# Autodesk Inventor assembly: centre wing
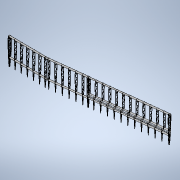
[picture p0: Inventor's stored thumbnail of the model, 180x180]
Saved by Autodesk Inventor 2022 (Build 260153000, 153)
## iProperties
Created: 2021-03-09
Part Number: centre wing
Document SubType Name: Assembly
Designer: Ferdinand Hubbard
Author: Ferdinand Hubbard
## Documents named in this file (15)
- C:\Users\Ferdinand Hubbard\Desktop\solarplane\cad\left wing section.iam
- C:\Users\Ferdinand Hubbard\Desktop\solarplane\cad\tubes\normal tubes\18mm tube.ipt
- C:\Users\Ferdinand Hubbard\Desktop\solarplane\cad\airfoils\full airfoil\full airfoil blueprint 19 mm.ipt
- C:\Users\Ferdinand Hubbard\Desktop\solarplane\cad\tubes\normal tubes\angle connector 19 mm.ipt
- C:\Users\Ferdinand Hubbard\Desktop\solarplane\cad\tubes\pre-aileron tubes\angle connector 19 mm.ipt
- C:\Users\Ferdinand Hubbard\Desktop\solarplane\cad\airfoils\full airfoil adjacent to aileron\full adjacent to aileron airfoil 19 mm big hole.ipt
- C:\Users\Ferdinand Hubbard\Desktop\solarplane\cad\tubes\normal tubes\15mm tube.ipt
- C:\Users\Ferdinand Hubbard\Desktop\solarplane\cad\tubes\normal tubes\7mm tube.ipt
- C:\Users\Ferdinand Hubbard\Desktop\solarplane\cad\tubes\normal tubes\straight connector aileron spar.ipt
- C:\Users\Ferdinand Hubbard\Desktop\solarplane\cad\airfoils\front half aileron\front half airfoil 16 mm.ipt
- C:\Users\Ferdinand Hubbard\Desktop\solarplane\cad\airfoils\full airfoil adjacent to aileron\full adjacent to aileron airfoil 19 mm small hole.ipt
- C:\Users\Ferdinand Hubbard\Desktop\solarplane\cad\airfoils\front half aileron\front half airfoil 19 mm.ipt
- C:\Users\Ferdinand Hubbard\Desktop\solarplane\cad\airfoils\back half aileron\back half aileron airfoil 19mm.ipt
- C:\Users\Ferdinand Hubbard\Desktop\solarplane\cad\tubes\back aileron tubes\18mm tube.ipt
- C:\Users\Ferdinand Hubbard\Desktop\solarplane\cad\tubes\back aileron tubes\15mm tube.ipt
## Components (57 placed, 11 different names)
1. 18mm tube:1 — Angle:2, Mate:10, Flush:2, Mate:25, Mate:26
2. 18mm tube:2 — Angle:1, Mate:11, Flush:1, Flush:3, Mate:27, Mate:28
3. full airfoil blueprint 19 mm:2 — Mate:1, Mate:2, Mate:3, Angle:1, Angle:2, Mate:10, Mate:11, Flush:1, Flush:2, Mate:21, Mate:22
4. full airfoil blueprint 19 mm:3 — Mate:1, Mate:2, Mate:3, Mate:7, Mate:8, Mate:9
5. full airfoil blueprint 19 mm:4 — Mate:7, Mate:8, Mate:9
6. full airfoil blueprint 19 mm:5 — Mate:18, Mate:19, Mate:20
7. full airfoil blueprint 19 mm:6 — Mate:18, Mate:19, Mate:20
8. full airfoil blueprint 19 mm:7
9. full airfoil blueprint 19 mm:8 — Mate:29, Mate:30
10. full airfoil blueprint 19 mm:9 — Flush:3, Mate:21, Mate:22
11. angle connector 19 mm:2 — Mate:25, Mate:26, Mate:29, Mate:49, Mate:51
12. angle connector 19 mm:3 — Mate:27, Mate:28, Mate:30, Mate:48, Mate:50, Mate:54
13. 18mm tube:3 — Mate:49, Mate:51, Mate:53, Mate:62, Flush:5
14. 18mm tube:4 — Mate:48, Mate:50, Mate:52, Mate:63, Mate:65
15. full airfoil blueprint 19 mm:11 — Mate:52, Mate:53, Mate:54
16. full airfoil blueprint 19 mm:12
17. full airfoil blueprint 19 mm:13
18. full airfoil blueprint 19 mm:14
19. full airfoil blueprint 19 mm:15 — Mate:55, Mate:56, Mate:57
20. full airfoil blueprint 19 mm:16 — Mate:55, Mate:56, Mate:57, Flush:4
21. full adjacent to aileron airfoil 19 mm small hole:1 — Mate:62, Flush:4, Flush:5, Mate:73, Angle:3, Flush:6, Flush:7, Angle:4, Mate:81, Mate:87, Mate:88, Mate:158, Mate:159, Flush:10, Mate:83
22. 18mm tube:6 — Mate:64, Mate:66, Mate:160
23. 15mm tube:1 — Mate:63, Mate:64, Mate:65, Mate:66
24. straight connector aileron spar:1 — Mate:74, Mate:75, Mate:76, Mate:77
25. 7mm tube:3 — Mate:75, Mate:77
26. 7mm tube:4 — Mate:73, Mate:74, Angle:3, Mate:76, Flush:6
27. 15mm tube:4 — Flush:7, Angle:4, Mate:79, Mate:86, Mate:87
28. 18mm tube:8 — Mate:79, Mate:86, Flush:12
29. front half airfoil 16 mm:1 — Mate:81, Mate:83, Mate:84, Mate:85, Mate:88, Mate:89
30. front half airfoil 16 mm:2 — Mate:84, Mate:85, Mate:89, Mate:93, Mate:94, Mate:95
31. front half airfoil 16 mm:3 — Mate:93, Mate:94, Mate:95
32. front half airfoil 16 mm:4 — Mate:99, Mate:100, Mate:101
33. front half airfoil 16 mm:5 — Mate:99, Mate:100, Mate:101
34. front half airfoil 16 mm:6 — Mate:111, Mate:112, Mate:113
35. front half airfoil 19 mm:1 — Mate:102, Mate:103, Mate:104, Mate:110, Mate:111, Mate:112, Mate:113
36. front half airfoil 19 mm:2 — Mate:102, Mate:103, Mate:104, Mate:108, Mate:109
37. front half airfoil 19 mm:3 — Mate:108, Mate:109, Mate:110
38. front half airfoil 19 mm:4 — Mate:117, Mate:118, Mate:119
39. front half airfoil 19 mm:5 — Mate:117, Mate:118, Mate:119
40. front half airfoil 19 mm:6 — Mate:163, Mate:164
41. back half aileron airfoil 19mm:1 — Mate:158, Flush:11, Mate:161
42. 18mm tube:9
43. 15mm tube:3
44. back half aileron airfoil 19mm:2
45. back half aileron airfoil 19mm:3
46. back half aileron airfoil 19mm:4
47. back half aileron airfoil 19mm:5
48. back half aileron airfoil 19mm:6
49. back half aileron airfoil 19mm:7
50. back half aileron airfoil 19mm:8
51. back half aileron airfoil 19mm:9
52. back half aileron airfoil 19mm:10
53. back half aileron airfoil 19mm:11
54. back half aileron airfoil 19mm:12
55. back half aileron airfoil 19mm:13 — Mate:159, Flush:10
56. full adjacent to aileron airfoil 19 mm big hole:1 — Mate:160, Flush:11, Mate:161, Flush:12, Mate:162
57. front half airfoil 19 mm:7 — Mate:162, Mate:163, Mate:164
## Relationships (160: Mate 143, Flush 12, Angle 5)
- Mate:1 (80 mm): full airfoil blueprint 19 mm:2 ↔ full airfoil blueprint 19 mm:3
- Mate:2: full airfoil blueprint 19 mm:2 ↔ full airfoil blueprint 19 mm:3
- Mate:3: full airfoil blueprint 19 mm:2 ↔ full airfoil blueprint 19 mm:3
- [Mate] (80 mm): full airfoil blueprint 19 mm:4 ↔ full airfoil blueprint 19 mm:5
- [Mate]: full airfoil blueprint 19 mm:4 ↔ full airfoil blueprint 19 mm:5
- [Mate]: full airfoil blueprint 19 mm:4 ↔ full airfoil blueprint 19 mm:5
- Mate:7: full airfoil blueprint 19 mm:3 ↔ full airfoil blueprint 19 mm:4
- Mate:8: full airfoil blueprint 19 mm:3 ↔ full airfoil blueprint 19 mm:4
- Mate:9 (80 mm): full airfoil blueprint 19 mm:3 ↔ full airfoil blueprint 19 mm:4
- Angle:1 (180 deg): 18mm tube:2 ↔ full airfoil blueprint 19 mm:2
- Angle:2 (180 deg): 18mm tube:1 ↔ full airfoil blueprint 19 mm:2
- Mate:10: 18mm tube:1 ↔ full airfoil blueprint 19 mm:2
- Mate:11: 18mm tube:2 ↔ full airfoil blueprint 19 mm:2
- Flush:1: 18mm tube:2 ↔ full airfoil blueprint 19 mm:2
- Flush:2: 18mm tube:1 ↔ full airfoil blueprint 19 mm:2
- [Mate]: full airfoil blueprint 19 mm:7 ↔ full airfoil blueprint 19 mm:8
- [Mate]: full airfoil blueprint 19 mm:7 ↔ full airfoil blueprint 19 mm:8
- [Mate]: full airfoil blueprint 19 mm:6 ↔ full airfoil blueprint 19 mm:7
- [Mate]: full airfoil blueprint 19 mm:6 ↔ full airfoil blueprint 19 mm:7
- [Mate] (80 mm): full airfoil blueprint 19 mm:6 ↔ full airfoil blueprint 19 mm:7
- Mate:18 (80 mm): full airfoil blueprint 19 mm:5 ↔ full airfoil blueprint 19 mm:6
- Mate:19: full airfoil blueprint 19 mm:5 ↔ full airfoil blueprint 19 mm:6
- Mate:20: full airfoil blueprint 19 mm:5 ↔ full airfoil blueprint 19 mm:6
- Flush:3 (10 mm): 18mm tube:2 ↔ full airfoil blueprint 19 mm:9
- Mate:21: full airfoil blueprint 19 mm:2 ↔ full airfoil blueprint 19 mm:9
- Mate:22: full airfoil blueprint 19 mm:2 ↔ full airfoil blueprint 19 mm:9
- Mate:25: 18mm tube:1 ↔ angle connector 19 mm:2
- Mate:26: 18mm tube:1 ↔ angle connector 19 mm:2
- Mate:27: 18mm tube:2 ↔ angle connector 19 mm:3
- Mate:28: 18mm tube:2 ↔ angle connector 19 mm:3
- Mate:29: full airfoil blueprint 19 mm:8 ↔ angle connector 19 mm:2
- Mate:30: full airfoil blueprint 19 mm:8 ↔ angle connector 19 mm:3
- [Mate] (80 mm): full airfoil blueprint 19 mm:12 ↔ full airfoil blueprint 19 mm:13
- [Mate]: full airfoil blueprint 19 mm:12 ↔ full airfoil blueprint 19 mm:13
- [Mate]: full airfoil blueprint 19 mm:12 ↔ full airfoil blueprint 19 mm:13
- [Mate]: full airfoil blueprint 19 mm:11 ↔ full airfoil blueprint 19 mm:12
- [Mate]: full airfoil blueprint 19 mm:11 ↔ full airfoil blueprint 19 mm:12
- [Mate] (80 mm): full airfoil blueprint 19 mm:11 ↔ full airfoil blueprint 19 mm:12
- [Mate]: full airfoil blueprint 19 mm:14 ↔ full airfoil blueprint 19 mm:15
- [Mate]: full airfoil blueprint 19 mm:14 ↔ full airfoil blueprint 19 mm:15
- [Mate] (80 mm): full airfoil blueprint 19 mm:14 ↔ full airfoil blueprint 19 mm:15
- [Mate] (80 mm): full airfoil blueprint 19 mm:13 ↔ full airfoil blueprint 19 mm:14
- [Mate]: full airfoil blueprint 19 mm:13 ↔ full airfoil blueprint 19 mm:14
- [Mate]: full airfoil blueprint 19 mm:13 ↔ full airfoil blueprint 19 mm:14
- Mate:48: angle connector 19 mm:3 ↔ 18mm tube:4
- Mate:49: angle connector 19 mm:2 ↔ 18mm tube:3
- Mate:50: angle connector 19 mm:3 ↔ 18mm tube:4
- Mate:51: angle connector 19 mm:2 ↔ 18mm tube:3
- Mate:52: 18mm tube:4 ↔ full airfoil blueprint 19 mm:11
- Mate:53: 18mm tube:3 ↔ full airfoil blueprint 19 mm:11
- Mate:54: angle connector 19 mm:3 ↔ full airfoil blueprint 19 mm:11
- Mate:55 (80 mm): full airfoil blueprint 19 mm:15 ↔ full airfoil blueprint 19 mm:16
- Mate:56: full airfoil blueprint 19 mm:15 ↔ full airfoil blueprint 19 mm:16
- Mate:57: full airfoil blueprint 19 mm:15 ↔ full airfoil blueprint 19 mm:16
- Mate:62: 18mm tube:3 ↔ full adjacent to aileron airfoil 19 mm small hole:1
- Flush:4: full airfoil blueprint 19 mm:16 ↔ full adjacent to aileron airfoil 19 mm small hole:1
- Mate:63: 18mm tube:4 ↔ 15mm tube:1
- Mate:64: 18mm tube:6 ↔ 15mm tube:1
- Mate:65: 18mm tube:4 ↔ 15mm tube:1
- Mate:66: 18mm tube:6 ↔ 15mm tube:1
- Flush:5: 18mm tube:3 ↔ full adjacent to aileron airfoil 19 mm small hole:1
- Mate:73: full adjacent to aileron airfoil 19 mm small hole:1 ↔ 7mm tube:4
- Mate:74: straight connector aileron spar:1 ↔ 7mm tube:4
- Mate:75: straight connector aileron spar:1 ↔ 7mm tube:3
- Angle:3 (180 deg): full adjacent to aileron airfoil 19 mm small hole:1 ↔ 7mm tube:4
- Mate:76: straight connector aileron spar:1 ↔ 7mm tube:4
- Mate:77: straight connector aileron spar:1 ↔ 7mm tube:3
- Flush:6 (8 mm): full adjacent to aileron airfoil 19 mm small hole:1 ↔ 7mm tube:4
- Flush:7 (1 mm): full adjacent to aileron airfoil 19 mm small hole:1 ↔ 15mm tube:4
- Angle:4 (180 deg): full adjacent to aileron airfoil 19 mm small hole:1 ↔ 15mm tube:4
- Mate:79: 15mm tube:4 ↔ 18mm tube:8
- Mate:81: full adjacent to aileron airfoil 19 mm small hole:1 ↔ front half airfoil 16 mm:1
- Mate:83 (12 mm): full adjacent to aileron airfoil 19 mm small hole:1 ↔ front half airfoil 16 mm:1
- Mate:84 (80 mm): front half airfoil 16 mm:1 ↔ front half airfoil 16 mm:2
- Mate:85: front half airfoil 16 mm:1 ↔ front half airfoil 16 mm:2
- Mate:86: 15mm tube:4 ↔ 18mm tube:8
- Mate:87: full adjacent to aileron airfoil 19 mm small hole:1 ↔ 15mm tube:4
- Mate:88: full adjacent to aileron airfoil 19 mm small hole:1 ↔ front half airfoil 16 mm:1
- Mate:89: front half airfoil 16 mm:1 ↔ front half airfoil 16 mm:2
- [Mate] (80 mm): front half airfoil 16 mm:3 ↔ front half airfoil 16 mm:4
- [Mate]: front half airfoil 16 mm:3 ↔ front half airfoil 16 mm:4
- [Mate]: front half airfoil 16 mm:3 ↔ front half airfoil 16 mm:4
- Mate:93 (80 mm): front half airfoil 16 mm:2 ↔ front half airfoil 16 mm:3
- Mate:94: front half airfoil 16 mm:2 ↔ front half airfoil 16 mm:3
- Mate:95: front half airfoil 16 mm:2 ↔ front half airfoil 16 mm:3
- [Mate] (80 mm): front half airfoil 16 mm:5 ↔ front half airfoil 16 mm:6
- [Mate]: front half airfoil 16 mm:5 ↔ front half airfoil 16 mm:6
- [Mate]: front half airfoil 16 mm:5 ↔ front half airfoil 16 mm:6
- Mate:99 (80 mm): front half airfoil 16 mm:4 ↔ front half airfoil 16 mm:5
- Mate:100: front half airfoil 16 mm:4 ↔ front half airfoil 16 mm:5
- Mate:101: front half airfoil 16 mm:4 ↔ front half airfoil 16 mm:5
- Mate:102 (80 mm): front half airfoil 19 mm:1 ↔ front half airfoil 19 mm:2
- Mate:103: front half airfoil 19 mm:1 ↔ front half airfoil 19 mm:2
- Mate:104: front half airfoil 19 mm:1 ↔ front half airfoil 19 mm:2
- [Mate] (80 mm): front half airfoil 19 mm:3 ↔ front half airfoil 19 mm:4
- [Mate]: front half airfoil 19 mm:3 ↔ front half airfoil 19 mm:4
- [Mate]: front half airfoil 19 mm:3 ↔ front half airfoil 19 mm:4
- Mate:108 (80 mm): front half airfoil 19 mm:2 ↔ front half airfoil 19 mm:3
- Mate:109: front half airfoil 19 mm:2 ↔ front half airfoil 19 mm:3
- Mate:110: front half airfoil 19 mm:1 ↔ front half airfoil 19 mm:3
- Mate:111 (80 mm): front half airfoil 16 mm:6 ↔ front half airfoil 19 mm:1
- Mate:112: front half airfoil 16 mm:6 ↔ front half airfoil 19 mm:1
- Mate:113: front half airfoil 16 mm:6 ↔ front half airfoil 19 mm:1
- [Mate] (80 mm): front half airfoil 19 mm:5 ↔ front half airfoil 19 mm:6
- [Mate]: front half airfoil 19 mm:5 ↔ front half airfoil 19 mm:6
- [Mate]: front half airfoil 19 mm:5 ↔ front half airfoil 19 mm:6
- Mate:117 (80 mm): front half airfoil 19 mm:4 ↔ front half airfoil 19 mm:5
- Mate:118: front half airfoil 19 mm:4 ↔ front half airfoil 19 mm:5
- Mate:119: front half airfoil 19 mm:4 ↔ front half airfoil 19 mm:5
- [Angle] (0 deg): back half aileron airfoil 19mm:1 ↔ 18mm tube:9
- [Mate]: back half aileron airfoil 19mm:1 ↔ 18mm tube:9
- [Flush] (1 mm): back half aileron airfoil 19mm:1 ↔ 18mm tube:9
- [Mate]: 18mm tube:9 ↔ 15mm tube:3
- [Mate]: 18mm tube:9 ↔ 15mm tube:3
- [Mate] (80 mm): back half aileron airfoil 19mm:1 ↔ back half aileron airfoil 19mm:2
- [Mate] (80 mm): back half aileron airfoil 19mm:2 ↔ back half aileron airfoil 19mm:3
- [Mate]: back half aileron airfoil 19mm:2 ↔ back half aileron airfoil 19mm:3
- [Mate]: back half aileron airfoil 19mm:2 ↔ back half aileron airfoil 19mm:3
- [Mate] (80 mm): back half aileron airfoil 19mm:4 ↔ back half aileron airfoil 19mm:5
- [Mate]: back half aileron airfoil 19mm:4 ↔ back half aileron airfoil 19mm:5
- [Mate]: back half aileron airfoil 19mm:4 ↔ back half aileron airfoil 19mm:5
- [Mate]: back half aileron airfoil 19mm:3 ↔ back half aileron airfoil 19mm:4
- [Mate] (80 mm): back half aileron airfoil 19mm:3 ↔ back half aileron airfoil 19mm:4
- [Mate]: back half aileron airfoil 19mm:3 ↔ back half aileron airfoil 19mm:4
- [Mate] (80 mm): back half aileron airfoil 19mm:6 ↔ back half aileron airfoil 19mm:7
- [Mate]: back half aileron airfoil 19mm:6 ↔ back half aileron airfoil 19mm:7
- [Mate]: back half aileron airfoil 19mm:6 ↔ back half aileron airfoil 19mm:7
- [Mate] (80 mm): back half aileron airfoil 19mm:8 ↔ back half aileron airfoil 19mm:9
- [Mate]: back half aileron airfoil 19mm:8 ↔ back half aileron airfoil 19mm:9
- [Mate]: back half aileron airfoil 19mm:8 ↔ back half aileron airfoil 19mm:9
- [Mate]: back half aileron airfoil 19mm:7 ↔ back half aileron airfoil 19mm:8
- [Mate] (80 mm): back half aileron airfoil 19mm:7 ↔ back half aileron airfoil 19mm:8
- [Mate]: back half aileron airfoil 19mm:7 ↔ back half aileron airfoil 19mm:8
- [Mate] (80 mm): back half aileron airfoil 19mm:5 ↔ back half aileron airfoil 19mm:6
- [Mate]: back half aileron airfoil 19mm:5 ↔ back half aileron airfoil 19mm:6
- [Mate]: back half aileron airfoil 19mm:5 ↔ back half aileron airfoil 19mm:6
- [Mate] (80 mm): back half aileron airfoil 19mm:11 ↔ back half aileron airfoil 19mm:12
- [Mate]: back half aileron airfoil 19mm:11 ↔ back half aileron airfoil 19mm:12
- [Mate]: back half aileron airfoil 19mm:11 ↔ back half aileron airfoil 19mm:12
- [Mate]: back half aileron airfoil 19mm:10 ↔ back half aileron airfoil 19mm:11
- [Mate] (80 mm): back half aileron airfoil 19mm:10 ↔ back half aileron airfoil 19mm:11
- [Mate]: back half aileron airfoil 19mm:10 ↔ back half aileron airfoil 19mm:11
- [Mate] (80 mm): back half aileron airfoil 19mm:9 ↔ back half aileron airfoil 19mm:10
- [Mate]: back half aileron airfoil 19mm:9 ↔ back half aileron airfoil 19mm:10
- [Mate]: back half aileron airfoil 19mm:9 ↔ back half aileron airfoil 19mm:10
- [Mate]: back half aileron airfoil 19mm:1 ↔ back half aileron airfoil 19mm:2
- [Mate]: back half aileron airfoil 19mm:1 ↔ back half aileron airfoil 19mm:2
- [Flush] (1 mm): 15mm tube:3 ↔ back half aileron airfoil 19mm:13
- [Mate]: back half aileron airfoil 19mm:12 ↔ back half aileron airfoil 19mm:13
- [Mate]: back half aileron airfoil 19mm:12 ↔ back half aileron airfoil 19mm:13
- Mate:158: full adjacent to aileron airfoil 19 mm small hole:1 ↔ back half aileron airfoil 19mm:1
- Mate:159 (4 mm): full adjacent to aileron airfoil 19 mm small hole:1 ↔ back half aileron airfoil 19mm:13
- Flush:10: full adjacent to aileron airfoil 19 mm small hole:1 ↔ back half aileron airfoil 19mm:13
- Mate:160: 18mm tube:6 ↔ full adjacent to aileron airfoil 19 mm big hole:1
- Flush:11: back half aileron airfoil 19mm:1 ↔ full adjacent to aileron airfoil 19 mm big hole:1
- Mate:161 (4 mm): back half aileron airfoil 19mm:1 ↔ full adjacent to aileron airfoil 19 mm big hole:1
- Flush:12 (1 mm): 18mm tube:8 ↔ full adjacent to aileron airfoil 19 mm big hole:1
- Mate:162 (1 mm): full adjacent to aileron airfoil 19 mm big hole:1 ↔ front half airfoil 19 mm:7
- Mate:163: front half airfoil 19 mm:6 ↔ front half airfoil 19 mm:7
- Mate:164: front half airfoil 19 mm:6 ↔ front half airfoil 19 mm:7
## Named parameters: d440_d437 = 80 mm, d441_d438 = 0 mm, d442_d439 = 0 mm, d453_d441_d438 = 0 mm, d454_d442_d439 = 0 mm, d455_d443 = 0 mm, d456_d444 = 0 mm, d457_d445 = 80 mm, d474_d455_d443 = 0 mm, d475_d456_d444 = 0 mm, d476_d457_d445 = 80 mm, d477_d458 = 80 mm, d478_d459 = 0 mm, d479_d460 = 0 mm, d486_d440_d437 = 80 mm, d487_d441_d438 = 0 mm, d488_d442_d439 = 0 mm, d489_d443 = 0 mm, d490_d444 = 0 mm, d491_d445 = 80 mm, d548_d541 = 80 mm, d549_d542 = 0 mm, d550_d547 = 0 mm, d554_d548_d541 = 80 mm, d555_d549_d542 = 0 mm, d556_d550_d547 = 0 mm, d563_d560 = 80 mm, d564_d561 = 0 mm, d565_d562 = 0 mm, d572_d563_d560 = 80 mm, d573_d564_d561 = 0 mm, d574_d565_d562 = 0 mm, d407_d398 = 80 mm, d408_d399 = 0 mm, d409_d400 = 0 mm, d410_d401_d398 = 80 mm, d411_d402_d399 = 0 mm, d412_d403_d400 = 0 mm, d413_d404 = 0 mm, d414_d405 = 80 mm, d415_d406 = 0 mm, d419_d410_d401_d398 = 80 mm, d420_d411_d402_d399 = 0 mm, d421_d412_d403_d400 = 0 mm, d422_d413_d404 = 0 mm, d423_d414_d405 = 80 mm, d424_d415_d406 = 0 mm, d401_d398 = 80 mm, d402_d399 = 0 mm, d403_d400 = 0 mm
